# Autodesk Inventor assembly: Сборка2
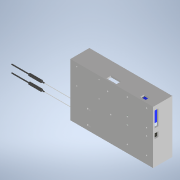
[picture p0: Inventor's stored thumbnail of the model, 180x180]
Saved by Autodesk Inventor 2022 (Build 260153000, 153)
## iProperties
Created: 2023-05-17
Part Number: Сборка2
Document SubType Name: Assembly
Designer: korsh624
Author: korsh624
## Documents named in this file (6)
- C:\Users\korsh624.VIRO\Desktop\модели\01062023\Сборка2.iam
- C:\Users\korsh624.VIRO\Desktop\модели\01062023\драйвер.ipt
- C:\Users\korsh624.VIRO\Desktop\модели\01062023\Receiver.ipt
- C:\Users\korsh624.VIRO\Desktop\модели\01062023\MEGA 2560 PRO (EMBED).iam
- C:\Users\korsh624.VIRO\Desktop\модели\01062023\2 Relay Module v2.ipt
- C:\Users\korsh624.VIRO\Desktop\модели\01062023\корпус.ipt
## Components (6 placed, 5 different names)
1. драйвер:1 — Заподлицо:1, Заподлицо:3, Заподлицо:5, Совмещение:1, Заподлицо:6, Заподлицо:8, Совмещение:2
2. драйвер:2 — Заподлицо:1, Совмещение:1, Заподлицо:6, Заподлицо:7, Заподлицо:10
3. Receiver:1 — Заподлицо:4, Заподлицо:8, Заподлицо:9
4. MEGA 2560 PRO (EMBED):1 [sub-assembly] — Заподлицо:5, Совмещение:2, Совмещение:3, Заподлицо:10
5. 2 Relay Module v2:1 — Заподлицо:3, Заподлицо:4, Заподлицо:7, Заподлицо:9, Совмещение:3, Заподлицо:11
6. корпус:1 — Заподлицо:11
## Relationships (13: Flush 10, Mate 3)
- Заподлицо:1 [Flush]: драйвер:1 ↔ драйвер:2
- Заподлицо:3 [Flush]: драйвер:1 ↔ 2 Relay Module v2:1
- Заподлицо:4 [Flush]: Receiver:1 ↔ 2 Relay Module v2:1
- Заподлицо:5 [Flush]: драйвер:1 ↔ MEGA 2560 PRO (EMBED):1
- Совмещение:1 [Mate] (5 mm): драйвер:1 ↔ драйвер:2
- Заподлицо:6 [Flush]: драйвер:1 ↔ драйвер:2
- Заподлицо:7 [Flush]: драйвер:2 ↔ 2 Relay Module v2:1
- Заподлицо:8 [Flush]: драйвер:1 ↔ Receiver:1
- Заподлицо:9 [Flush]: Receiver:1 ↔ 2 Relay Module v2:1
- Совмещение:2 [Mate] (5 mm): драйвер:1 ↔ MEGA 2560 PRO (EMBED):1
- Совмещение:3 [Mate] (5 mm): MEGA 2560 PRO (EMBED):1 ↔ 2 Relay Module v2:1
- Заподлицо:10 [Flush]: драйвер:2 ↔ MEGA 2560 PRO (EMBED):1
- Заподлицо:11 [Flush]: 2 Relay Module v2:1 ↔ корпус:1
